# Autodesk Inventor assembly: hotend
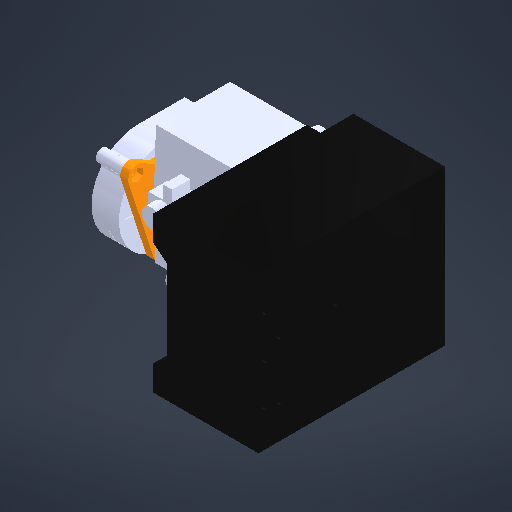
[picture p0: Inventor's stored thumbnail of the model, 512x512]
Saved by Autodesk Inventor 2025 (Build 290162000, 162)
## iProperties
Created: 2024-07-16
Part Number: hotend
Document SubType Name: Assembly
Designer: Windows 7 was better
Author: Windows 7 was better
## iProperties of the stored document Radial-Cooling-Fan-5015-DC12V.iam
Created: 2017-01-12
Part Number: Radial-Cooling-Fan-5015-DC12V
Description: STEP AP214
Document SubType Name: Assembly
Designer: Windows 7 was better
Sending System: SolidWorks 2016
Preprocessor: SwSTEP 2.0
Title: Radial-Cooling-Fan-5015-DC12V.STEP
Author: Ïîëüçîâàòåëü Windows
Revision Number: ANY
## iProperties of the stored document top.ipt
Created: 2024-07-17
Part Number: top
Material: Generic
Document SubType Name: Modeling
Designer: Windows 7 was better
Density: 1 g/cm^3
Appearance: Default
Author: Windows 7 was better
Revision Number: ANY
## iProperties of the stored document turbine.ipt
Created: 2024-07-17
Part Number: turbine
Material: Generic
Document SubType Name: Modeling
Designer: Windows 7 was better
Density: 1 g/cm^3
Appearance: Default
Author: Windows 7 was better
Revision Number: ANY
## iProperties of the stored document bottom.ipt
Created: 2024-07-17
Part Number: bottom
Material: Generic
Document SubType Name: Modeling
Designer: Windows 7 was better
Density: 1 g/cm^3
Appearance: Default
Author: Windows 7 was better
Revision Number: ANY
## Documents named in this file (11)
- C:\Users\Windows 7 was better\Documents\ReplicatorPlusConversion\CAD\hotend.iam
- C:\Users\Windows 7 was better\Documents\ReplicatorPlusConversion\CAD\makerbot-shroud.ipt
- C:\Users\Windows 7 was better\Documents\ReplicatorPlusConversion\CAD\hemera-mount.ipt
- C:\Users\Windows 7 was better\Documents\ReplicatorPlusConversion\CAD\hemera-xs-duct-mount-v2-eddy.ipt
- C:\Users\Windows 7 was better\Documents\ReplicatorPlusConversion\CAD\Hemera_XS_Reference_CAD.ipt
- **C:\Users\Windows 7 was better\Documents\ReplicatorPlusConversion\CAD\hotend.iam*LocalDocs*xAaaaq0aaAaaaaaaaAaaaahx0Ie*Radial-Cooling-Fan-5015-DC12V.iam
- C:\Users\Windows 7 was better\Documents\ReplicatorPlusConversion\CAD\eddy.ipt
- **C:\Users\Windows 7 was better\Documents\ReplicatorPlusConversion\CAD\hotend.iam*LocalDocs*xAaaaqgcaAaaaaaaaAaaaqsi4Lh*turbine.ipt
- **C:\Users\Windows 7 was better\Documents\ReplicatorPlusConversion\CAD\hotend.iam*LocalDocs*xAaaaagbaAaaaaaaaAaaaakrnTd*top.ipt
- **C:\Users\Windows 7 was better\Documents\ReplicatorPlusConversion\CAD\hotend.iam*LocalDocs*xAaaaqwbaAaaaaaaaAaaaqicgPe*bottom.ipt
- C:\Users\Windows 7 was better\Documents\makerbot stuff\Radial-Cooling-Fan-5015-DC12V.STEP
## Components (6 placed, 6 different names)
1. makerbot-shroud:1 — Flush:2
2. hemera-mount:1 — Flush:2
3. hemera-xs-duct-mount-v2-eddy:1
4. Hemera_XS_Reference_CAD:1
5. Radial-Cooling-Fan-5015-DC12V:1 [sub-assembly]
6. eddy:1
## Relationships (1: Flush 1)
- Flush:2: makerbot-shroud:1 ↔ hemera-mount:1
